# Autodesk Inventor assembly: keyboard-mockup_cherrymx
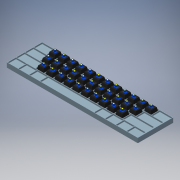
[picture p0: Inventor's stored thumbnail of the model, 180x180]
Saved by Autodesk Inventor 2016 (Build 200138000, 138)
## iProperties
Created: 2016-12-08
Part Number: keyboard-mockup_cherrymx
Document SubType Name: Assembly
Designer: Cemra JC
Author: Cemra JC
## Documents named in this file (4)
- J:\The Files\The Software Files\Projects\stenotoppers\cherrymx\mockup-parts\keyboard-mockup_cherrymx.iam
- J:\The Files\The Software Files\Projects\stenotoppers\cherrymx\mockup-parts\keyboard-base_standard.ipt
- J:\The Files\The Software Files\Projects\stenotoppers\cherrymx\mockup-parts\cherry-mx-switch\keyswitch_cherrymx.iam
- J:\The Files\The Software Files\Projects\stenotoppers\parameters.xlsx
## Components (34 placed, 2 different names)
1. keyboard-base_standard:1 — Rigid:1, Rigid:2, Rigid:3
2. keyswitch_cherrymx:1 [sub-assembly] — Rigid:1
3. keyswitch_cherrymx:4 [sub-assembly]
4. keyswitch_cherrymx:5 [sub-assembly]
5. keyswitch_cherrymx:6 [sub-assembly]
6. keyswitch_cherrymx:7 [sub-assembly]
7. keyswitch_cherrymx:8 [sub-assembly]
8. keyswitch_cherrymx:9 [sub-assembly]
9. keyswitch_cherrymx:10 [sub-assembly]
10. keyswitch_cherrymx:11 [sub-assembly]
11. keyswitch_cherrymx:12 [sub-assembly]
12. keyswitch_cherrymx:13 [sub-assembly]
13. keyswitch_cherrymx:14 [sub-assembly]
14. keyswitch_cherrymx:3 [sub-assembly] — Rigid:2
15. keyswitch_cherrymx:15 [sub-assembly]
16. keyswitch_cherrymx:16 [sub-assembly]
17. keyswitch_cherrymx:17 [sub-assembly]
18. keyswitch_cherrymx:18 [sub-assembly]
19. keyswitch_cherrymx:19 [sub-assembly]
20. keyswitch_cherrymx:20 [sub-assembly]
21. keyswitch_cherrymx:21 [sub-assembly]
22. keyswitch_cherrymx:22 [sub-assembly]
23. keyswitch_cherrymx:23 [sub-assembly]
24. keyswitch_cherrymx:24 [sub-assembly]
25. keyswitch_cherrymx:2 [sub-assembly] — Rigid:3
26. keyswitch_cherrymx:25 [sub-assembly]
27. keyswitch_cherrymx:26 [sub-assembly]
28. keyswitch_cherrymx:27 [sub-assembly]
29. keyswitch_cherrymx:28 [sub-assembly]
30. keyswitch_cherrymx:29 [sub-assembly]
31. keyswitch_cherrymx:30 [sub-assembly]
32. keyswitch_cherrymx:31 [sub-assembly]
33. keyswitch_cherrymx:32 [sub-assembly]
34. keyswitch_cherrymx:33 [sub-assembly]
## Component patterns: (12 elements, first: keyswitch_cherrymx:1), (11 elements, first: keyswitch_cherrymx:3), (10 elements, first: keyswitch_cherrymx:2)
## Relationships (3: WeldJoint 3)
- Rigid:1 [WeldJoint]: keyboard-base_standard:1 ↔ keyswitch_cherrymx:1
- Rigid:2 [WeldJoint]: keyboard-base_standard:1 ↔ keyswitch_cherrymx:3
- Rigid:3 [WeldJoint]: keyboard-base_standard:1 ↔ keyswitch_cherrymx:2
## Named parameters: k_width = 18 mm, k_height = 16.5 mm, k_height_low = 15 mm, k_taper_wide = 1.5 mm, k_taper_thin = 0.0001 mm, k_radius = 6 mm, k_wthick = 1.5 mm, k_ribthick = 1.5 mm, k_ribheight = 5 mm, k_poleoff = 2.25 mm, k_poledia = 5.3 mm, k_cmxw = 1.1 mm, k_cmxl = 4.15 mm, k_cmxd = 4 mm, k_shortening = 4.5 mm, s_bwidth = 14.4 mm, s_poleh = 3.6 mm, s_polebw = 5.4 mm, s_polebl = 7.45 mm, b_width = 285 mm, b_height = 77 mm, b_pad = 1 mm, b_tab = 27 mm, b_caps = 31.5 mm, b_lshift = 40.5 mm, b_rshift = 49.5 mm, b_ctrl = 22.5 mm, b_space = 117 mm, k_taper_side = 0.5 mm
